# Autodesk Inventor assembly: heater_bottom
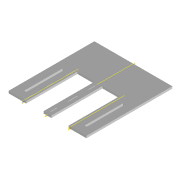
[picture p0: Inventor's stored thumbnail of the model, 180x180]
Saved by Autodesk Inventor 2020 (Build 240168000, 168)
## iProperties
Created: 2021-05-13
Part Number: heater_bottom
Document SubType Name: Assembly
Designer: Hsu Daniel
Author: Hsu Daniel
## Documents named in this file (4)
- D:\Daniel\NTU\makeNTU2021\大改\heater_bottom.iam
- D:\Daniel\NTU\makeNTU2021\大改\lr_bottom.ipt
- D:\Daniel\NTU\makeNTU2021\大改\mid_bottom.ipt
- D:\Daniel\NTU\makeNTU2021\大改\new_wire_bottom.ipt
## Components (4 placed, 3 different names)
1. lr_bottom:1 — Mate:2, Flush:6, Flush:7
2. lr_bottom:2 — Flush:5, Mate:3, Flush:8
3. mid_bottom:1 — Mate:1, Flush:1, Mate:4
4. new_wire_bottom:1 — Mate:1, Flush:1, Mate:2, Flush:6, Flush:5, Mate:3, Flush:7, Flush:8, Mate:4
## Relationships (9: Flush 5, Mate 4)
- Mate:1: mid_bottom:1 ↔ new_wire_bottom:1
- Flush:1: mid_bottom:1 ↔ new_wire_bottom:1
- Mate:2: lr_bottom:1 ↔ new_wire_bottom:1
- Flush:6: lr_bottom:1 ↔ new_wire_bottom:1
- Flush:5: lr_bottom:2 ↔ new_wire_bottom:1
- Mate:3: lr_bottom:2 ↔ new_wire_bottom:1
- Flush:7: lr_bottom:1 ↔ new_wire_bottom:1
- Flush:8: lr_bottom:2 ↔ new_wire_bottom:1
- Mate:4: mid_bottom:1 ↔ new_wire_bottom:1
